# Autodesk Inventor assembly: FullLegAssembly
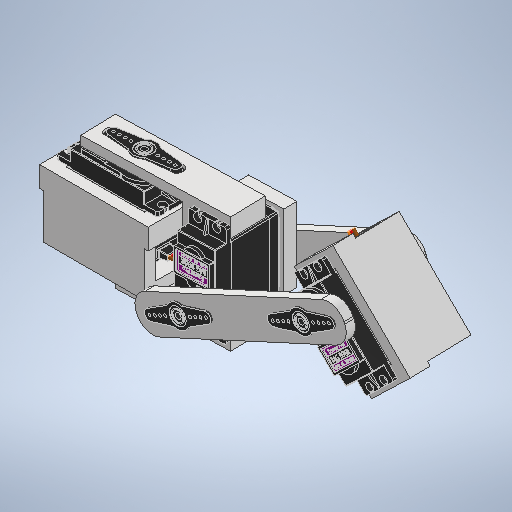
[picture p0: Inventor's stored thumbnail of the model, 512x512]
Saved by Autodesk Inventor 2025.1 (Build 291241020, 241B)
## iProperties
Created: 2024-09-10
Part Number: FullLegAssembly
Document SubType Name: Assembly
Designer: omiye
Author: omiye
## Documents named in this file (7)
- C:\Projects\Arduino\hexapod\legModels\FullLegAssembly.iam
- C:\Projects\Arduino\hexapod\legModels\MG996RServo.ipt
- C:\Projects\Arduino\hexapod\legModels\MG996RServoHolder.ipt
- C:\Projects\Arduino\hexapod\legModels\straightServoHorn.ipt
- C:\Projects\Arduino\hexapod\legModels\coxaModel.ipt
- C:\Projects\Arduino\hexapod\legModels\femurModel.ipt
- C:\Projects\Arduino\hexapod\legModels\tibiaModel.ipt
## Components (10 placed, 6 different names)
1. MG996RServo:1 — Mate:1, Mate:2, Mate:5, Mate:6, Mate:9, Mate:10, Mate:11, Mate:12
2. MG996RServoHolder:1 — Mate:1, Mate:2, Mate:9, Mate:10, Mate:11, Mate:12
3. straightServoHorn:1 — Mate:5, Mate:6, Mate:13, Mate:14, Mate:15, Mate:16
4. coxaModel:1 — Mate:13, Mate:14, Mate:15, Mate:16, Mate:17, Mate:18, Mate:19, Mate:20
5. MG996RServo:2 — Mate:17, Mate:18, Mate:19, Mate:20, Mate:21, Mate:22
6. straightServoHorn:2 — Mate:21, Mate:22, Mate:32, Mate:33, Mate:34
7. MG996RServo:3 — Mate:30, Mate:31, Mate:36, Mate:38, Mate:39, Mate:40, Mate:41, Mate:42, Mate:43
8. straightServoHorn:3 — Mate:30, Mate:31, Mate:35, Mate:37
9. femurModel:1 — Mate:32, Mate:33, Mate:34, Mate:35, Mate:36, Mate:37
10. tibiaModel:1 — Mate:38, Mate:39, Mate:40, Mate:41, Mate:42, Mate:43
## Relationships (32: Mate 32)
- Mate:1: MG996RServo:1 ↔ MG996RServoHolder:1
- Mate:2: MG996RServo:1 ↔ MG996RServoHolder:1
- Mate:5: MG996RServo:1 ↔ straightServoHorn:1
- Mate:6: MG996RServo:1 ↔ straightServoHorn:1
- Mate:9: MG996RServo:1 ↔ MG996RServoHolder:1
- Mate:10: MG996RServo:1 ↔ MG996RServoHolder:1
- Mate:11: MG996RServo:1 ↔ MG996RServoHolder:1
- Mate:12: MG996RServo:1 ↔ MG996RServoHolder:1
- Mate:13: straightServoHorn:1 ↔ coxaModel:1
- Mate:14: straightServoHorn:1 ↔ coxaModel:1
- Mate:15: straightServoHorn:1 ↔ coxaModel:1
- Mate:16: straightServoHorn:1 ↔ coxaModel:1
- Mate:17: coxaModel:1 ↔ MG996RServo:2
- Mate:18: coxaModel:1 ↔ MG996RServo:2
- Mate:19: coxaModel:1 ↔ MG996RServo:2
- Mate:20: coxaModel:1 ↔ MG996RServo:2
- Mate:21: MG996RServo:2 ↔ straightServoHorn:2
- Mate:22: MG996RServo:2 ↔ straightServoHorn:2
- Mate:30: MG996RServo:3 ↔ straightServoHorn:3
- Mate:31: MG996RServo:3 ↔ straightServoHorn:3
- Mate:32: straightServoHorn:2 ↔ femurModel:1
- Mate:33: straightServoHorn:2 ↔ femurModel:1
- Mate:34: straightServoHorn:2 ↔ femurModel:1
- Mate:35: straightServoHorn:3 ↔ femurModel:1
- Mate:36: MG996RServo:3 ↔ femurModel:1
- Mate:37: straightServoHorn:3 ↔ femurModel:1
- Mate:38: MG996RServo:3 ↔ tibiaModel:1
- Mate:39: MG996RServo:3 ↔ tibiaModel:1
- Mate:40: MG996RServo:3 ↔ tibiaModel:1
- Mate:41: MG996RServo:3 ↔ tibiaModel:1
- Mate:42: MG996RServo:3 ↔ tibiaModel:1
- Mate:43: MG996RServo:3 ↔ tibiaModel:1
